# Autodesk Inventor assembly: CyberducksRobot
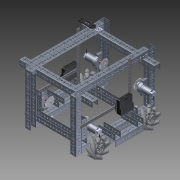
[picture p0: Inventor's stored thumbnail of the model, 180x180]
Saved by Autodesk Inventor 2015 (Build 190159000, 159)
## iProperties
Created: 2014-11-17
Part Number: CyberducksRobot
Document SubType Name: Assembly
Designer: Evan
Author: Evan
## Documents named in this file (20)
- C:\Users\Evan\Desktop\Final cad ftc\CyberducksRobot.iam
- C:\Users\Evan\Desktop\Final cad ftc\Tetrix_Kit - Ring_it_up\Tetrix_Kit_FTC\Imported Components\tetrix_739069_2012_416_channel\tetrix_739069_2012_416_channel.ipt
- C:\Users\Evan\Desktop\Final cad ftc\Tetrix_Kit - Ring_it_up\Tetrix_Kit_FTC\Imported Components\tetrix_739091_2012\tetrix_739091_2012.ipt
- C:\Users\Evan\Desktop\Final cad ftc\Tetrix_Kit - Ring_it_up\Tetrix_Kit_FTC\Imported Components\tetrix_739068_2012_288_channel\tetrix_739068_2012_288_channel.ipt
- C:\Users\Evan\Desktop\Final cad ftc\step onliune\Imported Components\Pitsco Education-739270\Pitsco Education-739270.ipt
- C:\Users\Evan\Desktop\Final cad ftc\Tetrix_Kit - Ring_it_up\Tetrix_Kit_FTC\Imported Components\tetrix_739066_2012_96_channel\tetrix_739066_2012_96_channel.ipt
- C:\Users\Evan\Desktop\Final cad ftc\Tetrix_Kit - Ring_it_up\Tetrix_Kit_FTC\Imported Components\tetrix_739067_2012_160_channel\tetrix_739067_2012_160_channel.ipt
- C:\Users\Evan\Desktop\Final cad ftc\Tetrix_Kit - Ring_it_up\Tetrix_Kit_FTC\Imported Components\tetrix_739088_2012\tetrix_739088_2012.ipt
- C:\Users\Evan\Desktop\Final cad ftc\Tetrix_Kit - Ring_it_up\Imported Components\276-1447\276-1447.iam
- C:\Users\Evan\Desktop\Final cad ftc\Tetrix_Kit - Ring_it_up\Tetrix_Kit_FTC\Imported Components\tetrix_739089_2012\tetrix_739089_2012.ipt
- C:\Users\Evan\Desktop\Final cad ftc\Tetrix_Kit - Ring_it_up\Tetrix_Kit_FTC\Imported Components\tetrix_739083_2012\tetrix_739083_2012.iam
- C:\Users\Evan\Desktop\Final cad ftc\Tetrix_Kit - Ring_it_up\Tetrix_Kit_FTC\Imported Components\tetrix_739079_2012\tetrix_739079_2012.iam
- C:\Users\Evan\Desktop\Final cad ftc\Tetrix_Kit - Ring_it_up\Tetrix_Kit_FTC\Imported Components\tetrix_739169_2012\tetrix_739169_2012.ipt
- C:\Users\Evan\Desktop\Final cad ftc\Tetrix_Kit - Ring_it_up\Tetrix_Kit_FTC\Imported Components\tetrix_739172_2012\tetrix_739172_2012.iam
- C:\Users\Evan\Desktop\Final cad ftc\Tetrix_Kit - Ring_it_up\Tetrix_Kit_FTC\Imported Components\tetrix_739165_2012\tetrix_739165_2012.ipt
- C:\Users\Evan\Desktop\Final cad ftc\Tetrix_Kit - Ring_it_up\Tetrix_Kit_FTC\Imported Components\tetrix_739070_2012\tetrix_739070_2012.ipt
- C:\Users\Evan\Desktop\Final cad ftc\Assembly2.iam
- C:\Users\Evan\Desktop\Final cad ftc\Tetrix_Kit - Ring_it_up\Tetrix_Kit_FTC\Imported Components\tetrix_991444_2012\tetrix_991444_2012.ipt
- C:\Users\Evan\Desktop\Final cad ftc\Tetrix_Kit - Ring_it_up\Tetrix_Kit_FTC\Imported Components\tetrix_739176_2012\tetrix_739176_2012.ipt
- C:\Users\Evan\Desktop\Final cad ftc\Tetrix_Kit - Ring_it_up\Tetrix_Kit_FTC\Imported Components\tetrix_731903_2012\tetrix_731903_2012.ipt
## Components (70 placed, 19 different names)
1. tetrix_739069_2012_416_channel:1 — Insert:3, Insert:4, Insert:7, Insert:8, Mate:1, Mate:4, Mate:5, Mate:12, Mate:20
2. tetrix_739069_2012_416_channel:2 — Insert:1, Insert:2, Insert:5, Insert:6, Mate:2, Mate:3, Mate:6, Mate:11, Mate:16
3. tetrix_739091_2012:1 — Insert:1, Insert:15
4. tetrix_739091_2012:2 — Insert:2, Insert:16
5. tetrix_739091_2012:3 — Insert:4
6. tetrix_739091_2012:4 — Insert:3
7. tetrix_739091_2012:5 — Insert:5
8. tetrix_739091_2012:6 — Insert:7, Insert:14
9. tetrix_739091_2012:7 — Insert:8, Insert:13
10. tetrix_739091_2012:8 — Insert:6
11. tetrix_739068_2012_288_channel:1 — Mate:1, Mate:2, Mate:52, Mate:53
12. tetrix_739068_2012_288_channel:2 — Mate:3, Mate:4, Mate:17, Mate:18
13. Pitsco Education-739270:1 — Mate:5, Mate:51
14. Pitsco Education-739270:2 — Mate:6, Mate:50
15. tetrix_739066_2012_96_channel:1 — Mate:12, Mate:13, Mate:18
16. tetrix_739066_2012_96_channel:2 — Mate:19, Mate:20
17. tetrix_739066_2012_96_channel:3 — Mate:11, Mate:14, Mate:17
18. tetrix_739066_2012_96_channel:4 — Mate:15, Mate:16
19. tetrix_739067_2012_160_channel:1 — Mate:14, Mate:15
20. tetrix_739067_2012_160_channel:2 — Mate:13, Mate:19
21. tetrix_739088_2012:3 — Insert:11, Insert:13, Insert:28
22. tetrix_739088_2012:4 — Insert:9, Insert:15, Insert:25
23. 276-1447:1 [sub-assembly] — Insert:11
24. 276-1447:3 [sub-assembly] — Insert:9
25. tetrix_739088_2012:5 — Insert:16, Insert:26
26. 276-1447:5 [sub-assembly]
27. tetrix_739088_2012:6 — Insert:14, Insert:27
28. 276-1447:6 [sub-assembly]
29. tetrix_739066_2012_96_channel:5 — Mate:35, Mate:57
30. tetrix_739089_2012:1 — Mate:35, Insert:20
31. tetrix_739089_2012:3 — Insert:19
32. tetrix_739089_2012:4 — Insert:17
33. tetrix_739083_2012:1 [sub-assembly] — Insert:19, Insert:23, Insert:33
34. tetrix_739083_2012:2 [sub-assembly] — Insert:20, Insert:24, Insert:34
35. tetrix_739083_2012:3 [sub-assembly] — Insert:17, Insert:21, Insert:31
36. tetrix_739079_2012:2 [sub-assembly] — Insert:21, Mate:39
37. tetrix_739079_2012:3 [sub-assembly] — Insert:23, Mate:40
38. tetrix_739079_2012:4 [sub-assembly] — Insert:24, Mate:42
39. tetrix_739169_2012:1 — Mate:40
40. tetrix_739169_2012:2 — Mate:42
41. tetrix_739169_2012:3 — Mate:39
42. tetrix_739172_2012:1 [sub-assembly] — Insert:25, Mate:43
43. tetrix_739172_2012:2 [sub-assembly] — Insert:26, Mate:46
44. tetrix_739165_2012:1 — Mate:43
45. tetrix_739165_2012:2 — Mate:46
46. tetrix_739165_2012:3 — Mate:45
47. tetrix_739165_2012:4 — Mate:44
48. tetrix_739172_2012:3 [sub-assembly] — Insert:27, Mate:45
49. tetrix_739172_2012:4 [sub-assembly] — Insert:28, Mate:44
50. tetrix_739070_2012:1 — Mate:56
51. tetrix_739070_2012:2 — Mate:57
52. tetrix_739070_2012:3 — Mate:58, Mate:61
53. tetrix_739070_2012:4 — Mate:59, Mate:60
54. tetrix_739089_2012:5 — Mate:48, Insert:29
55. tetrix_739079_2012:5 [sub-assembly] — Insert:30, Mate:49
56. tetrix_739169_2012:5 — Mate:49
57. tetrix_739083_2012:5 [sub-assembly] — Insert:29, Insert:30, Insert:32
58. tetrix_739066_2012_96_channel:7 — Mate:48, Mate:56
59. Assembly2:1 [sub-assembly] — Mate:54, Mate:55, Mate:58, Mate:59, Mate:62
60. tetrix_739068_2012_288_channel:3 — Mate:53
61. tetrix_739068_2012_288_channel:4 — Mate:50, Mate:55
62. tetrix_739068_2012_288_channel:5 — Mate:52, Mate:54
63. tetrix_739068_2012_288_channel:6 — Mate:51
64. tetrix_991444_2012:1 — Mate:60
65. tetrix_991444_2012:2 — Mate:61
66. tetrix_739176_2012:1 — Mate:62
67. tetrix_731903_2012:1 — Insert:31
68. tetrix_731903_2012:2 — Insert:32
69. tetrix_731903_2012:3 — Insert:34
70. tetrix_731903_2012:4 — Insert:33
## Relationships (71: Mate 39, Insert 32)
- Insert:1: tetrix_739069_2012_416_channel:2 ↔ tetrix_739091_2012:1
- Insert:2: tetrix_739069_2012_416_channel:2 ↔ tetrix_739091_2012:2
- Insert:3: tetrix_739069_2012_416_channel:1 ↔ tetrix_739091_2012:4
- Insert:4: tetrix_739069_2012_416_channel:1 ↔ tetrix_739091_2012:3
- Insert:5: tetrix_739069_2012_416_channel:2 ↔ tetrix_739091_2012:5
- Insert:6: tetrix_739069_2012_416_channel:2 ↔ tetrix_739091_2012:8
- Insert:7: tetrix_739069_2012_416_channel:1 ↔ tetrix_739091_2012:6
- Insert:8: tetrix_739069_2012_416_channel:1 ↔ tetrix_739091_2012:7
- Mate:1: tetrix_739069_2012_416_channel:1 ↔ tetrix_739068_2012_288_channel:1
- Mate:2: tetrix_739069_2012_416_channel:2 ↔ tetrix_739068_2012_288_channel:1
- Mate:3: tetrix_739069_2012_416_channel:2 ↔ tetrix_739068_2012_288_channel:2
- Mate:4: tetrix_739069_2012_416_channel:1 ↔ tetrix_739068_2012_288_channel:2
- Mate:5: tetrix_739069_2012_416_channel:1 ↔ Pitsco Education-739270:1
- Mate:6: tetrix_739069_2012_416_channel:2 ↔ Pitsco Education-739270:2
- Mate:11: tetrix_739069_2012_416_channel:2 ↔ tetrix_739066_2012_96_channel:3
- Mate:12: tetrix_739069_2012_416_channel:1 ↔ tetrix_739066_2012_96_channel:1
- Mate:13: tetrix_739066_2012_96_channel:1 ↔ tetrix_739067_2012_160_channel:2
- Mate:14: tetrix_739066_2012_96_channel:3 ↔ tetrix_739067_2012_160_channel:1
- Mate:15: tetrix_739066_2012_96_channel:4 ↔ tetrix_739067_2012_160_channel:1
- Mate:16: tetrix_739069_2012_416_channel:2 ↔ tetrix_739066_2012_96_channel:4
- Mate:17: tetrix_739068_2012_288_channel:2 ↔ tetrix_739066_2012_96_channel:3
- Mate:18: tetrix_739068_2012_288_channel:2 ↔ tetrix_739066_2012_96_channel:1
- Mate:19: tetrix_739066_2012_96_channel:2 ↔ tetrix_739067_2012_160_channel:2
- Mate:20: tetrix_739069_2012_416_channel:1 ↔ tetrix_739066_2012_96_channel:2
- Insert:9 (-25.4 mm): tetrix_739088_2012:4 ↔ 276-1447:3
- [Insert] (-25.4 mm): tetrix_739088_2012:5 ↔ 276-1447:5
- Insert:11 (-25.4 mm): tetrix_739088_2012:3 ↔ 276-1447:1
- [Insert] (-25.4 mm): tetrix_739088_2012:6 ↔ 276-1447:6
- Insert:13 (-57.15 mm): tetrix_739091_2012:7 ↔ tetrix_739088_2012:3
- Insert:14 (-57.15 mm): tetrix_739091_2012:6 ↔ tetrix_739088_2012:6
- Insert:15 (-57.15 mm): tetrix_739091_2012:1 ↔ tetrix_739088_2012:4
- Insert:16 (-57.15 mm): tetrix_739091_2012:2 ↔ tetrix_739088_2012:5
- Mate:35: tetrix_739066_2012_96_channel:5 ↔ tetrix_739089_2012:1
- Insert:17 (-19.05 mm): tetrix_739089_2012:4 ↔ tetrix_739083_2012:3
- Insert:19 (-19.05 mm): tetrix_739089_2012:3 ↔ tetrix_739083_2012:1
- Insert:20 (-19.05 mm): tetrix_739089_2012:1 ↔ tetrix_739083_2012:2
- Insert:21 (19.05 mm): tetrix_739083_2012:3 ↔ tetrix_739079_2012:2
- Insert:23 (-12.7 mm): tetrix_739083_2012:1 ↔ tetrix_739079_2012:3
- Insert:24 (-12.7 mm): tetrix_739083_2012:2 ↔ tetrix_739079_2012:4
- Mate:39: tetrix_739079_2012:2 ↔ tetrix_739169_2012:3
- Mate:40: tetrix_739079_2012:3 ↔ tetrix_739169_2012:1
- Mate:42: tetrix_739079_2012:4 ↔ tetrix_739169_2012:2
- Insert:25 (-19.05 mm): tetrix_739088_2012:4 ↔ tetrix_739172_2012:1
- Insert:26 (-19.05 mm): tetrix_739088_2012:5 ↔ tetrix_739172_2012:2
- Mate:43: tetrix_739172_2012:1 ↔ tetrix_739165_2012:1
- Insert:27 (-10.16 mm): tetrix_739088_2012:6 ↔ tetrix_739172_2012:3
- Insert:28 (-10.16 mm): tetrix_739088_2012:3 ↔ tetrix_739172_2012:4
- Mate:44: tetrix_739165_2012:4 ↔ tetrix_739172_2012:4
- Mate:45: tetrix_739165_2012:3 ↔ tetrix_739172_2012:3
- Mate:46: tetrix_739172_2012:2 ↔ tetrix_739165_2012:2
- Mate:48: tetrix_739089_2012:5 ↔ tetrix_739066_2012_96_channel:7
- Insert:29 (-13.97 mm): tetrix_739089_2012:5 ↔ tetrix_739083_2012:5
- Insert:30 (-19.05 mm): tetrix_739079_2012:5 ↔ tetrix_739083_2012:5
- Mate:49: tetrix_739079_2012:5 ↔ tetrix_739169_2012:5
- Mate:50: Pitsco Education-739270:2 ↔ tetrix_739068_2012_288_channel:4
- Mate:51: Pitsco Education-739270:1 ↔ tetrix_739068_2012_288_channel:6
- Mate:52: tetrix_739068_2012_288_channel:1 ↔ tetrix_739068_2012_288_channel:5
- Mate:53: tetrix_739068_2012_288_channel:1 ↔ tetrix_739068_2012_288_channel:3
- Mate:54: Assembly2:1 ↔ tetrix_739068_2012_288_channel:5
- Mate:55: Assembly2:1 ↔ tetrix_739068_2012_288_channel:4
- Mate:56: tetrix_739070_2012:1 ↔ tetrix_739066_2012_96_channel:7
- Mate:57: tetrix_739066_2012_96_channel:5 ↔ tetrix_739070_2012:2
- Mate:58: tetrix_739070_2012:3 ↔ Assembly2:1
- Mate:59: tetrix_739070_2012:4 ↔ Assembly2:1
- Mate:60: tetrix_739070_2012:4 ↔ tetrix_991444_2012:1
- Mate:61: tetrix_739070_2012:3 ↔ tetrix_991444_2012:2
- Mate:62: Assembly2:1 ↔ tetrix_739176_2012:1
- Insert:31: tetrix_739083_2012:3 ↔ tetrix_731903_2012:1
- Insert:32: tetrix_739083_2012:5 ↔ tetrix_731903_2012:2
- Insert:33: tetrix_739083_2012:1 ↔ tetrix_731903_2012:4
- Insert:34: tetrix_739083_2012:2 ↔ tetrix_731903_2012:3
## Named parameters: d41_d40 = -25.4 mm, d43_d42 = -25.4 mm
